# Autodesk Inventor assembly: Nema 17 Stepper Motor
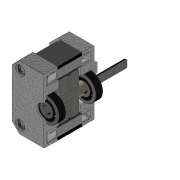
[picture p0: Inventor's stored thumbnail of the model, 180x180]
Saved by Autodesk Inventor 2020.2 (Build 242310000, 310)
## iProperties
Created: 2020-01-17
Part Number: Nema 17 Stepper Motor
Document SubType Name: Assembly
Designer: james
Mass: 221.621 g
Surface Area: 516.91 cm^2
Volume: 44.7637 cm^3
Density: 4.95091 g/cm^3
Author: james
## Documents named in this file (17)
- D:\Users\James B\Documents\Beech Projects\3D scanner\CAD\Shared Components\Bought Parts\Stepper Motor\Nema 17 Stepper Motor.iam
- D:\Users\James B\Documents\Beech Projects\3D scanner\CAD\Shared Components\Bought Parts\Stepper Motor\Nema 17 Top Cap.ipt
- T:\ContentCentre\en-US\BS 3469(2)\BS 3469 - 02 - 5 x 16 x 5.ipt
- D:\Users\James B\Documents\Beech Projects\3D scanner\CAD\Shared Components\Bought Parts\Stepper Motor\Nema 17 Plastic Spacer 2.ipt
- D:\Users\James B\Documents\Beech Projects\3D scanner\CAD\Shared Components\Bought Parts\Stepper Motor\Nema 17 Plastic Spacer 1.ipt
- D:\Users\James B\Documents\Beech Projects\3D scanner\CAD\Shared Components\Bought Parts\Stepper Motor\Nema 17 shaft.ipt
- T:\ContentCentre\en-US\ANSI B27.7(1)\ANSI B27.7 - 53.9(1).ipt
- D:\Users\James B\Documents\Beech Projects\3D scanner\CAD\Shared Components\Bought Parts\Stepper Motor\Nema 17 Base Cap.ipt
- D:\Users\James B\Documents\Beech Projects\3D scanner\CAD\Shared Components\Bought Parts\Stepper Motor\Nema 17 Central Spacer.ipt
- D:\Users\James B\Documents\Beech Projects\3D scanner\CAD\Shared Components\Bought Parts\Stepper Motor\Nema 17 Stator Face.ipt
- D:\Users\James B\Documents\Beech Projects\3D scanner\CAD\Shared Components\Bought Parts\Stepper Motor\Nema 17 plastic.ipt
- D:\Users\James B\Documents\Beech Projects\3D scanner\CAD\Shared Components\Bought Parts\Stepper Motor\S6B-PH-K-S.ipt
- T:\ContentCentre\en-US\SS-EN-ISO 7045  H\EN ISO 7045 - M3 x 25H.ipt
- D:\Users\James B\Documents\Beech Projects\3D scanner\CAD\Shared Components\Bought Parts\Stepper Motor\Nema 17 Coil.ipt
- D:\Users\James B\Documents\Beech Projects\3D scanner\CAD\Shared Components\Bought Parts\Stepper Motor\Nema 17 plastic protector.ipt
- D:\Users\James B\Documents\Beech Projects\3D scanner\CAD\Shared Components\Bought Parts\Stepper Motor\Nema 17 PCB.ipt
- D:\Users\James B\Documents\Beech Projects\3D scanner\CAD\Shared Components\Bought Parts\Stepper Motor\Nema 17 Sprung Washer.ipt
## Components (27 placed, 16 different names)
1. Nema 17 Top Cap:1 — Mate:2, Mate:3, Mate:4, Mate:17, Mate:18
2. BS 3469 (Metric) 02 - 5 x 16 x 5:1 — Insert:5, Mate:3
3. BS 3469 (Metric) 02 - 5 x 16 x 5:2 — Insert:1, Insert:7
4. Nema 17 Plastic Spacer 2:1 — Insert:3
5. Nema 17 Plastic Spacer 1:1 — Insert:4, Insert:5
6. Nema 17 shaft:1 — Insert:1, Mate:1, Insert:2, Insert:4
7. E-Ring 5:1 — Mate:1, Insert:2, Insert:3
8. Nema 17 Base Cap:1 — Insert:7, Mate:2, Mate:4, Insert:8, Mate:5, Mate:6, Flush:4, Insert:9, Insert:10, Insert:11, Insert:12, Mate:12, Mate:13, Angle:2
9. Nema 17 Central Spacer:1 — Insert:8, Mate:5, Flush:1, Mate:7, Mate:8, Flush:3, Flush:5
10. Nema 17 Stator Face:1 — Flush:1, Mate:6, Flush:2
11. Nema 17 plastic:1 — Mate:7, Mate:8, Flush:3, Mate:10, Mate:11, Angle:1, Mate:14
12. S6B-PH-K-S:1 — Flush:4, Mate:9, Flush:5, Mate:15, Mate:16
13. SS EN ISO 7045 H M3 x 25:1 — Insert:10
14. SS EN ISO 7045 H M3 x 25:2 — Insert:11
15. SS EN ISO 7045 H M3 x 25:3 — Insert:9
16. SS EN ISO 7045 H M3 x 25:4 — Insert:12
17. Nema 17 plastic protector:1 — Mate:12, Mate:13, Angle:2
18. Nema 17 PCB:1 — Mate:14, Mate:15, Mate:16
19. Nema 17 Sprung Washer:1 — Mate:17, Mate:18
20. Nema 17 Coil:1 — Mate:10, Mate:11, Angle:1
21. Nema 17 Coil:2
22. Nema 17 Coil:3
23. Nema 17 Coil:4
24. Nema 17 Coil:5
25. Nema 17 Coil:6
26. Nema 17 Coil:7
27. Nema 17 Coil:8
## Component patterns: (8 elements, first: Nema 17 Coil:1)
## Relationships (36: Mate 18, Insert 11, Flush 5, Angle 2)
- Insert:1: BS 3469 (Metric) 02 - 5 x 16 x 5:2 ↔ Nema 17 shaft:1
- Mate:1: Nema 17 shaft:1 ↔ E-Ring 5:1
- Insert:2: Nema 17 shaft:1 ↔ E-Ring 5:1
- Insert:3: Nema 17 Plastic Spacer 2:1 ↔ E-Ring 5:1
- Insert:4: Nema 17 Plastic Spacer 1:1 ↔ Nema 17 shaft:1
- Insert:5: BS 3469 (Metric) 02 - 5 x 16 x 5:1 ↔ Nema 17 Plastic Spacer 1:1
- Insert:7: BS 3469 (Metric) 02 - 5 x 16 x 5:2 ↔ Nema 17 Base Cap:1
- Mate:2: Nema 17 Top Cap:1 ↔ Nema 17 Base Cap:1
- Mate:3: Nema 17 Top Cap:1 ↔ BS 3469 (Metric) 02 - 5 x 16 x 5:1
- Mate:4 (16 mm): Nema 17 Top Cap:1 ↔ Nema 17 Base Cap:1
- Insert:8: Nema 17 Base Cap:1 ↔ Nema 17 Central Spacer:1
- Mate:5: Nema 17 Base Cap:1 ↔ Nema 17 Central Spacer:1
- Flush:1: Nema 17 Central Spacer:1 ↔ Nema 17 Stator Face:1
- Mate:6: Nema 17 Base Cap:1 ↔ Nema 17 Stator Face:1
- Flush:2: Nema 17 Stator Face:1
- Mate:7: Nema 17 Central Spacer:1 ↔ Nema 17 plastic:1
- Mate:8: Nema 17 Central Spacer:1 ↔ Nema 17 plastic:1
- Flush:3 (-4.35 mm): Nema 17 Central Spacer:1 ↔ Nema 17 plastic:1
- Flush:4 (-0.5 mm): Nema 17 Base Cap:1 ↔ S6B-PH-K-S:1
- Mate:9: S6B-PH-K-S:1
- Flush:5 (-6 mm): Nema 17 Central Spacer:1 ↔ S6B-PH-K-S:1
- Insert:9: Nema 17 Base Cap:1 ↔ SS EN ISO 7045 H M3 x 25:3
- Insert:10: Nema 17 Base Cap:1 ↔ SS EN ISO 7045 H M3 x 25:1
- Insert:11: Nema 17 Base Cap:1 ↔ SS EN ISO 7045 H M3 x 25:2
- Insert:12: Nema 17 Base Cap:1 ↔ SS EN ISO 7045 H M3 x 25:4
- Mate:10: Nema 17 plastic:1 ↔ Nema 17 Coil:1
- Mate:11: Nema 17 plastic:1 ↔ Nema 17 Coil:1
- Angle:1 (180 deg): Nema 17 plastic:1 ↔ Nema 17 Coil:1
- Mate:12: Nema 17 Base Cap:1 ↔ Nema 17 plastic protector:1
- Mate:13: Nema 17 Base Cap:1 ↔ Nema 17 plastic protector:1
- Angle:2 (0 deg): Nema 17 Base Cap:1 ↔ Nema 17 plastic protector:1
- Mate:14: Nema 17 plastic:1 ↔ Nema 17 PCB:1
- Mate:15: S6B-PH-K-S:1 ↔ Nema 17 PCB:1
- Mate:16: S6B-PH-K-S:1 ↔ Nema 17 PCB:1
- Mate:17: Nema 17 Top Cap:1 ↔ Nema 17 Sprung Washer:1
- Mate:18: Nema 17 Top Cap:1 ↔ Nema 17 Sprung Washer:1
